# Autodesk Inventor assembly: DMP_counterweight_Assembly
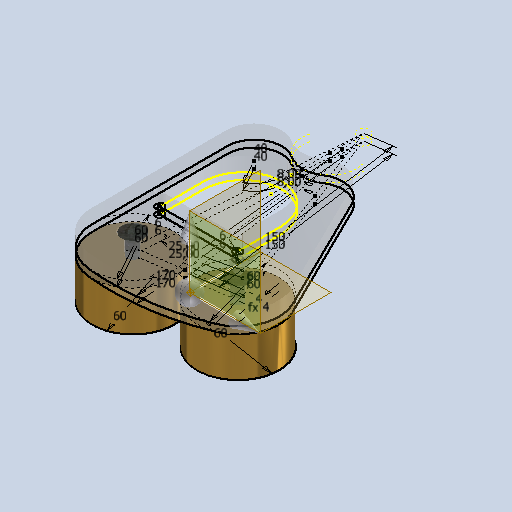
[picture p0: Inventor's stored thumbnail of the model, 512x512]
Saved by Autodesk Inventor 2024 (Build 280153000, 153)
## iProperties
Created: 2022-11-02
Part Number: DMP_counterweight_Assembly
Document SubType Name: Assembly
Designer: alexw
Mass: 1649.56 g
Surface Area: 894.843 cm^2
Volume: 352.297 cm^3
Density: 4.6823 g/cm^3
Author: alexw
## Documents named in this file (7)
- C:\Users\AEWALDER\Documents\Inventor\03_CurrentProjects\MasterThesis\PSM_V1_Rillenkugellager\DMP_counterweight_Assembly.iam
- C:\Users\AEWALDER\Documents\Inventor\03_CurrentProjects\MasterThesis\PSM_V1_Rillenkugellager\DPMAxis1_Weights.ipt
- C:\Users\AEWALDER\Documents\Inventor\03_CurrentProjects\MasterThesis\PSM_V1_Rillenkugellager\DPM_Counterweight_Fixation.ipt
- C:\Users\AEWALDER\Documents\Inventor\03_CurrentProjects\MasterThesis\PSM_V1_Rillenkugellager\ContentCenter\de-DE\ISO 10642(1)\ISO 10642 - M8 x  60.ipt
- C:\Users\AEWALDER\Documents\Inventor\03_CurrentProjects\MasterThesis\PSM_V1_Rillenkugellager\DPM_Counterweight_Fixation_DistanceDisc.ipt
- C:\Users\AEWALDER\Documents\Inventor\03_CurrentProjects\MasterThesis\PSM_V1_Rillenkugellager\ContentCenter\de-DE\ISO 7092\ISO 7092 - ST 8 - 140 HV.ipt
- C:\Users\AEWALDER\Documents\Inventor\03_CurrentProjects\MasterThesis\PSM_V1_Rillenkugellager\ContentCenter\de-DE\ISO 4032(2)\ISO 4032 - M8 - ISO.ipt
## Components (10 placed, 6 different names)
1. DPM_Counterweight_Fixation:1 — Passend:7, Passend:8, Passend:9, Fluchtend:1, Fluchtend:2, Fluchtend:3, Tangential:1, Tangential:2, Passend:24, Passend:25
2. DPMAxis1_Weights:1 — Passend:11, Passend:13, Passend:23
3. DPMAxis1_Weights:2 — Passend:10, Passend:15, Passend:22, Passend:24
4. ISO 10642 M8x60:1 — Passend:14, Passend:18, Tangential:1, Passend:22
5. ISO 10642 M8x60:2 — Passend:12, Passend:16, Tangential:2, Passend:23, Passend:25
6. DPM_Counterweight_Fixation_DistanceDisc:1 — Passend:7, Passend:8, Passend:9, Passend:10, Passend:11
7. ISO 7092 ST 8 - 140 HV:1 — Passend:12, Passend:13, Passend:17
8. ISO 7092 ST 8 - 140 HV:2 — Passend:14, Passend:15, Passend:19
9. ISO 4032 M8:1 — Passend:16, Passend:17
10. ISO 4032 M8:2 — Passend:18, Passend:19
## Relationships (22: Mate 17, Flush 3, Tangent 2)
- Passend:7 [Mate]: DPM_Counterweight_Fixation:1 ↔ DPM_Counterweight_Fixation_DistanceDisc:1
- Passend:8 [Mate]: DPM_Counterweight_Fixation:1 ↔ DPM_Counterweight_Fixation_DistanceDisc:1
- Passend:9 [Mate]: DPM_Counterweight_Fixation:1 ↔ DPM_Counterweight_Fixation_DistanceDisc:1
- Passend:10 [Mate]: DPMAxis1_Weights:2 ↔ DPM_Counterweight_Fixation_DistanceDisc:1
- Passend:11 [Mate]: DPMAxis1_Weights:1 ↔ DPM_Counterweight_Fixation_DistanceDisc:1
- Fluchtend:1 [Flush]: DPM_Counterweight_Fixation:1
- Fluchtend:2 [Flush]: DPM_Counterweight_Fixation:1
- Fluchtend:3 [Flush]: DPM_Counterweight_Fixation:1
- Passend:12 [Mate]: ISO 10642 M8x60:2 ↔ ISO 7092 ST 8 - 140 HV:1
- Passend:13 [Mate]: DPMAxis1_Weights:1 ↔ ISO 7092 ST 8 - 140 HV:1
- Passend:14 [Mate]: ISO 10642 M8x60:1 ↔ ISO 7092 ST 8 - 140 HV:2
- Passend:15 [Mate]: DPMAxis1_Weights:2 ↔ ISO 7092 ST 8 - 140 HV:2
- Passend:16 [Mate]: ISO 10642 M8x60:2 ↔ ISO 4032 M8:1
- Passend:17 [Mate]: ISO 7092 ST 8 - 140 HV:1 ↔ ISO 4032 M8:1
- Passend:18 [Mate]: ISO 10642 M8x60:1 ↔ ISO 4032 M8:2
- Passend:19 [Mate]: ISO 7092 ST 8 - 140 HV:2 ↔ ISO 4032 M8:2
- Tangential:1: DPM_Counterweight_Fixation:1 ↔ ISO 10642 M8x60:1
- Tangential:2: DPM_Counterweight_Fixation:1 ↔ ISO 10642 M8x60:2
- Passend:22 [Mate]: DPMAxis1_Weights:2 ↔ ISO 10642 M8x60:1
- Passend:23 [Mate]: DPMAxis1_Weights:1 ↔ ISO 10642 M8x60:2
- Passend:24 [Mate]: DPM_Counterweight_Fixation:1 ↔ DPMAxis1_Weights:2
- Passend:25 [Mate]: DPM_Counterweight_Fixation:1 ↔ ISO 10642 M8x60:2
